# Autodesk Inventor assembly: mould_top_p2
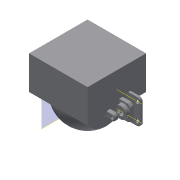
[picture p0: Inventor's stored thumbnail of the model, 180x180]
Saved by Autodesk Inventor 2017 (Build 210142000, 142)
## iProperties
Created: 2018-06-07
Part Number: mould_top_p2
Document SubType Name: Assembly
Designer: Nic
Author: Nic
## Documents named in this file (3)
- C:\Users\Nic\Documents\Antenna\mould_top_p2.iam
- C:\Users\Nic\Documents\Antenna\mould_top_proc1.ipt
- C:\Users\Nic\Documents\Antenna\mould_casing.ipt
## Components (2 placed, 2 different names)
1. mould_top_proc1:1 — Ball:1, Angle:1, Angle:2
2. mould_casing:1 — Ball:1, Angle:1, Angle:2
## Relationships (3: Angle 2, BallJoint 1)
- Ball:1: mould_top_proc1:1 ↔ mould_casing:1
- Angle:1 (0 deg): mould_top_proc1:1 ↔ mould_casing:1
- Angle:2 (0 deg): mould_top_proc1:1 ↔ mould_casing:1
